# Autodesk Inventor assembly: SecondJoint
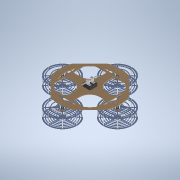
[picture p0: Inventor's stored thumbnail of the model, 180x180]
Saved by Autodesk Inventor 2021 (Build 250183000, 183)
## iProperties
Created: 2023-10-17
Part Number: SecondJoint
Document SubType Name: Assembly
Designer: Lenovo
Mass: 1997.94 g
Surface Area: 9056.95 cm^2
Volume: 1354.83 cm^3
Density: 1.47468 g/cm^3
Author: Lenovo
## Documents named in this file (12)
- E:\0 semester 10\GP2\2DOF_Hover\CAD\Workspaces\Workspace\SecondJoint.iam
- E:\0 semester 10\GP2\2DOF_Hover\CAD\Workspaces\Workspace\Assembly231015Kerangka Bawah 1.ipt
- E:\0 semester 10\GP2\2DOF_Hover\CAD\Workspaces\Workspace\shaft.ipt
- E:\0 semester 10\GP2\2DOF_Hover\CAD\Workspaces\Workspace\Holder Tube-R8.ipt
- E:\0 semester 10\GP2\2DOF_Hover\CAD\Workspaces\Workspace\Part15.ipt
- E:\0 semester 10\GP2\2DOF_Hover\CAD\Workspaces\Workspace\Assembly1.iam
- E:\0 semester 10\GP2\2DOF_Hover\CAD\Workspaces\Workspace\Libraries\Content Center Files\en-US\BS EN ISO 4015\BS EN ISO 4015 - M3x20.ipt
- E:\0 semester 10\GP2\2DOF_Hover\CAD\Workspaces\Workspace\Libraries\Content Center Files\en-US\AS 1112 (4)\AS 1112 - M3(2).ipt
- E:\0 semester 10\GP2\2DOF_Hover\CAD\Workspaces\Workspace\Libraries\Content Center Files\en-US\ISO 4034(2)\ISO 4034 - M5 - ISO.ipt
- E:\0 semester 10\GP2\2DOF_Hover\CAD\Libraries\Content Center Files\en-US\ISO 4015\ISO 4015 - M5 x 45.ipt
- E:\0 semester 10\GP2\2DOF_Hover\CAD\Workspaces\Workspace\pcb.ipt
- E:\0 semester 10\GP2\2DOF_Hover\CAD\Workspaces\Workspace\9. Fan.ipt
## Components (42 placed, 11 different names)
1. Kerangka Bawah 1_10 — Flush:2, Flush:3, Mate:55, Mate:56, Mate:57, Mate:78, Mate:79, Mate:80, Mate:81, Mate:82, Mate:83, Mate:84, Mate:85, Mate:86, Mate:87, Mate:88, Mate:89, Insert:1, Insert:2, Insert:3, Insert:4, Insert:5, Insert:6, Insert:7, Insert:8, Insert:9, Insert:10, Insert:11, Insert:12, Insert:13, Insert:14, Insert:15, Insert:16, Angle:2, Angle:3, Angle:4, Angle:5, Angle:6, Angle:7, Angle:8, Angle:9, Angle:10, Angle:11, Angle:12, Angle:13, Angle:14, Angle:15, Angle:16, Angle:17, Insert:21, Mate:111, Mate:112, Mate:113, Flush:6, Flush:7, Mate:122
2. Holder Tube-R8:1 — Mate:50, Mate:54, Mate:98, Mate:99, Angle:19, Mate:100, Mate:101, Mate:109, Mate:110, Flush:122, Mate:123
3. Holder Tube-R8:2 — Angle:1, Mate:47, Mate:53, Angle:22, Mate:102, Mate:103, Mate:105, Mate:106, Mate:107, Mate:108
4. shaft:1 — Angle:1, Mate:53, Mate:54, Mate:123
5. Part15:1 — Flush:2, Flush:3, Mate:47, Mate:50, Mate:55, Mate:56, Mate:57, Mate:100, Mate:101, Mate:102, Mate:103, Mate:124, Mate:125
6. Assembly1:1 [sub-assembly] — Mate:78, Mate:79, Mate:80, Insert:17, Insert:18, Insert:19, Insert:20, Mate:119, Flush:10
7. Assembly1:2 [sub-assembly] — Mate:84, Mate:85, Mate:86, Flush:121, Mate:121
8. Assembly1:3 [sub-assembly] — Mate:87, Mate:88, Mate:89, Mate:117, Flush:8
9. Assembly1:4 [sub-assembly] — Mate:81, Mate:82, Mate:83, Flush:9, Mate:118
10. pcb:1 — Flush:6, Flush:7, Mate:122
11. 9. Fan:1 — Mate:117, Flush:8
12. 9. Fan:2 — Flush:9, Mate:118
13. 9. Fan:3 — Mate:119, Flush:10
14. 9. Fan:4 — Flush:121, Mate:121
15. ISO 4015 M5 x 45:2 — Mate:105, Mate:106, Mate:115
16. ISO 4034 M5:2 — Mate:111, Mate:114
17. ISO 4015 M5 x 45:3 — Mate:107, Mate:108, Mate:116
18. ISO 4034 M5:3 — Mate:112, Mate:115
19. ISO 4015 M5 x 45:4 — Mate:109, Mate:110, Mate:114
20. ISO 4034 M5:4 — Mate:113, Mate:116
21. BS EN ISO 4015 M3x20:1 — Insert:1, Angle:2
22. BS EN ISO 4015 M3x20:2 — Insert:2, Angle:15
23. BS EN ISO 4015 M3x20:3 — Insert:3, Angle:4
24. BS EN ISO 4015 M3x20:4 — Insert:4, Angle:6
25. BS EN ISO 4015 M3x20:5 — Insert:5, Angle:12
26. BS EN ISO 4015 M3x20:6 — Insert:6, Angle:13
27. BS EN ISO 4015 M3x20:7 — Insert:7, Angle:7
28. BS EN ISO 4015 M3x20:8 — Insert:8, Angle:14
29. BS EN ISO 4015 M3x20:9 — Insert:9, Angle:17
30. BS EN ISO 4015 M3x20:10 — Insert:10, Angle:3
31. BS EN ISO 4015 M3x20:11 — Insert:11, Angle:8
32. BS EN ISO 4015 M3x20:12 — Insert:12, Angle:11
33. BS EN ISO 4015 M3x20:13 — Insert:13, Angle:10
34. BS EN ISO 4015 M3x20:14 — Insert:14, Angle:9
35. BS EN ISO 4015 M3x20:15 — Insert:15, Angle:5
36. BS EN ISO 4015 M3x20:16 — Insert:16, Angle:16
37. AS 1112 (4) - Metric M3:1 — Insert:17
38. AS 1112 (4) - Metric M3:2 — Insert:18
39. AS 1112 (4) - Metric M3:3 — Insert:19
40. AS 1112 (4) - Metric M3:4 — Insert:20
41. ISO 4015 M5 x 45:1 — Mate:98, Mate:99, Angle:19
42. ISO 4034 M5:1 — Insert:21, Angle:22
## Relationships (94: Mate 45, Insert 21, Angle 19, Flush 9)
- Angle:1 (0 deg): Holder Tube-R8:2 ↔ shaft:1
- Flush:2: Kerangka Bawah 1_10 ↔ Part15:1
- Flush:3: Kerangka Bawah 1_10 ↔ Part15:1
- Mate:47: Holder Tube-R8:2 ↔ Part15:1
- Mate:50: Holder Tube-R8:1 ↔ Part15:1
- Mate:53: Holder Tube-R8:2 ↔ shaft:1
- Mate:54: Holder Tube-R8:1 ↔ shaft:1
- Mate:55: Kerangka Bawah 1_10 ↔ Part15:1
- Mate:56: Kerangka Bawah 1_10 ↔ Part15:1
- Mate:57: Kerangka Bawah 1_10 ↔ Part15:1
- Mate:78 (30 mm): Kerangka Bawah 1_10 ↔ Assembly1:1
- Mate:79: Kerangka Bawah 1_10 ↔ Assembly1:1
- Mate:80: Kerangka Bawah 1_10 ↔ Assembly1:1
- Mate:81: Kerangka Bawah 1_10 ↔ Assembly1:4
- Mate:82: Kerangka Bawah 1_10 ↔ Assembly1:4
- Mate:83 (30 mm): Kerangka Bawah 1_10 ↔ Assembly1:4
- Mate:84: Kerangka Bawah 1_10 ↔ Assembly1:2
- Mate:85: Kerangka Bawah 1_10 ↔ Assembly1:2
- Mate:86 (30 mm): Kerangka Bawah 1_10 ↔ Assembly1:2
- Mate:87: Kerangka Bawah 1_10 ↔ Assembly1:3
- Mate:88: Kerangka Bawah 1_10 ↔ Assembly1:3
- Mate:89 (30 mm): Kerangka Bawah 1_10 ↔ Assembly1:3
- Insert:1: Kerangka Bawah 1_10 ↔ BS EN ISO 4015 M3x20:1
- Insert:2: Kerangka Bawah 1_10 ↔ BS EN ISO 4015 M3x20:2
- Insert:3: Kerangka Bawah 1_10 ↔ BS EN ISO 4015 M3x20:3
- Insert:4: Kerangka Bawah 1_10 ↔ BS EN ISO 4015 M3x20:4
- Insert:5: Kerangka Bawah 1_10 ↔ BS EN ISO 4015 M3x20:5
- Insert:6: Kerangka Bawah 1_10 ↔ BS EN ISO 4015 M3x20:6
- Insert:7: Kerangka Bawah 1_10 ↔ BS EN ISO 4015 M3x20:7
- Insert:8: Kerangka Bawah 1_10 ↔ BS EN ISO 4015 M3x20:8
- Insert:9: Kerangka Bawah 1_10 ↔ BS EN ISO 4015 M3x20:9
- Insert:10: Kerangka Bawah 1_10 ↔ BS EN ISO 4015 M3x20:10
- Insert:11: Kerangka Bawah 1_10 ↔ BS EN ISO 4015 M3x20:11
- Insert:12: Kerangka Bawah 1_10 ↔ BS EN ISO 4015 M3x20:12
- Insert:13: Kerangka Bawah 1_10 ↔ BS EN ISO 4015 M3x20:13
- Insert:14: Kerangka Bawah 1_10 ↔ BS EN ISO 4015 M3x20:14
- Insert:15: Kerangka Bawah 1_10 ↔ BS EN ISO 4015 M3x20:15
- Insert:16: Kerangka Bawah 1_10 ↔ BS EN ISO 4015 M3x20:16
- Insert:17: Assembly1:1 ↔ AS 1112 (4) - Metric M3:1
- Insert:18: Assembly1:1 ↔ AS 1112 (4) - Metric M3:2
- Insert:19: Assembly1:1 ↔ AS 1112 (4) - Metric M3:3
- Insert:20: Assembly1:1 ↔ AS 1112 (4) - Metric M3:4
- Angle:2 (0 deg): Kerangka Bawah 1_10 ↔ BS EN ISO 4015 M3x20:1
- Angle:3 (0 deg): Kerangka Bawah 1_10 ↔ BS EN ISO 4015 M3x20:10
- Angle:4 (0 deg): Kerangka Bawah 1_10 ↔ BS EN ISO 4015 M3x20:3
- Angle:5 (0 deg): Kerangka Bawah 1_10 ↔ BS EN ISO 4015 M3x20:15
- Angle:6 (0 deg): Kerangka Bawah 1_10 ↔ BS EN ISO 4015 M3x20:4
- Angle:7 (0 deg): Kerangka Bawah 1_10 ↔ BS EN ISO 4015 M3x20:7
- Angle:8 (0 deg): Kerangka Bawah 1_10 ↔ BS EN ISO 4015 M3x20:11
- Angle:9 (0 deg): Kerangka Bawah 1_10 ↔ BS EN ISO 4015 M3x20:14
- Angle:10 (0 deg): Kerangka Bawah 1_10 ↔ BS EN ISO 4015 M3x20:13
- Angle:11 (0 deg): Kerangka Bawah 1_10 ↔ BS EN ISO 4015 M3x20:12
- Angle:12 (0 deg): Kerangka Bawah 1_10 ↔ BS EN ISO 4015 M3x20:5
- Angle:13 (0 deg): Kerangka Bawah 1_10 ↔ BS EN ISO 4015 M3x20:6
- Angle:14 (0 deg): Kerangka Bawah 1_10 ↔ BS EN ISO 4015 M3x20:8
- Angle:15 (0 deg): Kerangka Bawah 1_10 ↔ BS EN ISO 4015 M3x20:2
- Angle:16 (0 deg): Kerangka Bawah 1_10 ↔ BS EN ISO 4015 M3x20:16
- Angle:17 (0 deg): Kerangka Bawah 1_10 ↔ BS EN ISO 4015 M3x20:9
- Mate:98: Holder Tube-R8:1 ↔ ISO 4015 M5 x 45:1
- Mate:99: Holder Tube-R8:1 ↔ ISO 4015 M5 x 45:1
- Angle:19 (0 deg): Holder Tube-R8:1 ↔ ISO 4015 M5 x 45:1
- Insert:21: Kerangka Bawah 1_10 ↔ ISO 4034 M5:1
- Angle:22 (0 deg): Holder Tube-R8:2 ↔ ISO 4034 M5:1
- Mate:100: Holder Tube-R8:1 ↔ Part15:1
- Mate:101: Holder Tube-R8:1 ↔ Part15:1
- Mate:102: Holder Tube-R8:2 ↔ Part15:1
- Mate:103: Holder Tube-R8:2 ↔ Part15:1
- Mate:105: Holder Tube-R8:2 ↔ ISO 4015 M5 x 45:2
- Mate:106: Holder Tube-R8:2 ↔ ISO 4015 M5 x 45:2
- Mate:107: Holder Tube-R8:2 ↔ ISO 4015 M5 x 45:3
- Mate:108: Holder Tube-R8:2 ↔ ISO 4015 M5 x 45:3
- Mate:109: Holder Tube-R8:1 ↔ ISO 4015 M5 x 45:4
- Mate:110: Holder Tube-R8:1 ↔ ISO 4015 M5 x 45:4
- Mate:111: Kerangka Bawah 1_10 ↔ ISO 4034 M5:2
- Mate:112: Kerangka Bawah 1_10 ↔ ISO 4034 M5:3
- Mate:113: Kerangka Bawah 1_10 ↔ ISO 4034 M5:4
- Mate:114: ISO 4034 M5:2 ↔ ISO 4015 M5 x 45:4
- Mate:115: ISO 4015 M5 x 45:2 ↔ ISO 4034 M5:3
- Mate:116: ISO 4015 M5 x 45:3 ↔ ISO 4034 M5:4
- Flush:6: Kerangka Bawah 1_10 ↔ pcb:1
- Flush:7: Kerangka Bawah 1_10 ↔ pcb:1
- Mate:117: Assembly1:3 ↔ 9. Fan:1
- Flush:8: Assembly1:3 ↔ 9. Fan:1
- Flush:9: Assembly1:4 ↔ 9. Fan:2
- Mate:118: Assembly1:4 ↔ 9. Fan:2
- Mate:119: Assembly1:1 ↔ 9. Fan:3
- Flush:10: Assembly1:1 ↔ 9. Fan:3
- Flush:121: Assembly1:2 ↔ 9. Fan:4
- Mate:121: Assembly1:2 ↔ 9. Fan:4
- Mate:122: Kerangka Bawah 1_10 ↔ pcb:1
- Flush:122: Holder Tube-R8:1
- Mate:123 (-43 mm): Holder Tube-R8:1 ↔ shaft:1
- Mate:124 (-30 mm): Part15:1
- Mate:125 (-30 mm): Part15:1
